# Autodesk Inventor assembly: CameraUnit
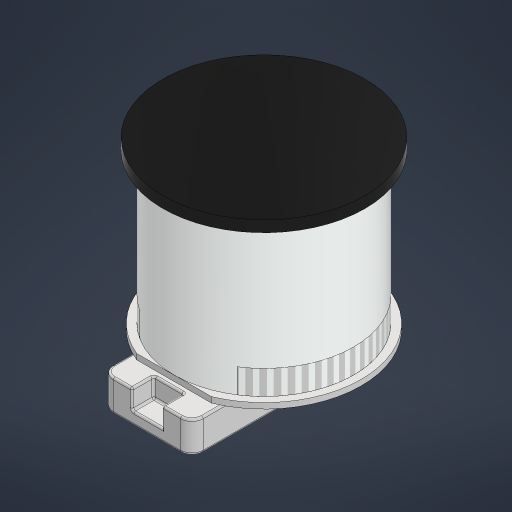
[picture p0: Inventor's stored thumbnail of the model, 512x512]
Saved by Autodesk Inventor 2024.2 (Build 282272000, 272)
## iProperties
Created: 2023-12-21
Part Number: CameraUnit
Document SubType Name: Assembly
Designer: Hanaoka
Author: Hanaoka
## Documents named in this file (5)
- G:\共有ドライブ\reRo\05_個人\hanaoka\inventor\CameraUnit.iam
- G:\共有ドライブ\reRo\05_個人\hanaoka\inventor\Camera_pipe.ipt
- G:\共有ドライブ\reRo\05_個人\hanaoka\inventor\Camera_mirror.ipt
- G:\共有ドライブ\reRo\05_個人\hanaoka\inventor\UnitV_OV7740_M12.ipt
- G:\共有ドライブ\reRo\05_個人\hanaoka\inventor\Mirror_Mount.ipt
## Components (4 placed, 4 different names)
1. Camera_pipe:1 — メイト:1, メイト:2, メイト:3, メイト:4
2. Camera_mirror:1 — メイト:1, メイト:2
3. UnitV_OV7740_M12:1 — フラッシュ:1, フラッシュ:2, フラッシュ:3
4. Mirror_Mount:1 — フラッシュ:1, フラッシュ:2, フラッシュ:3, メイト:3, メイト:4
## Relationships (7: Mate 4, Flush 3)
- メイト:1 [Mate]: Camera_pipe:1 ↔ Camera_mirror:1
- メイト:2 [Mate]: Camera_pipe:1 ↔ Camera_mirror:1
- フラッシュ:1 [Flush]: UnitV_OV7740_M12:1 ↔ Mirror_Mount:1
- フラッシュ:2 [Flush]: UnitV_OV7740_M12:1 ↔ Mirror_Mount:1
- フラッシュ:3 [Flush]: UnitV_OV7740_M12:1 ↔ Mirror_Mount:1
- メイト:3 [Mate]: Camera_pipe:1 ↔ Mirror_Mount:1
- メイト:4 [Mate]: Camera_pipe:1 ↔ Mirror_Mount:1
